# Autodesk Inventor assembly: 1_6RadiusPole_WithBolt_AJB
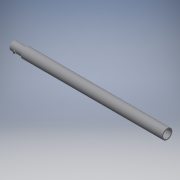
[picture p0: Inventor's stored thumbnail of the model, 180x180]
Saved by Autodesk Inventor 2018 (Build 220112000, 112)
## iProperties
Created: 2018-02-03
Part Number: 1_6RadiusPole_WithBolt_AJB
Document SubType Name: Assembly
Designer: Alec temporary
Author: Alec temporary
## Documents named in this file (3)
- M:\TPS\9th Grade\CADD 2017-2018\Current\Ferris Wheel Group Project\Group Project Week 2b\Alec\1_6RadiusPole_WithBolt_AJB.iam
- M:\TPS\9th Grade\CADD 2017-2018\Current\Ferris Wheel Group Project\Group Project Week 2b\Alec\1_6RadiusPoleAJB.ipt
- M:\TPS\9th Grade\CADD 2017-2018\Current\Ferris Wheel Group Project\Group Project Week 2b\Alec\HexBoltAJB.ipt
## Components (2 placed, 2 different names)
1. 1_6RadiusPoleAJB:1 — Mate:2, Tangent:1
2. HexBoltAJB:2 — Mate:2, Tangent:1
## Relationships (2: Mate 1, Tangent 1)
- Mate:2: 1_6RadiusPoleAJB:1 ↔ HexBoltAJB:2
- Tangent:1: 1_6RadiusPoleAJB:1 ↔ HexBoltAJB:2
